# Autodesk Inventor assembly: Assembly
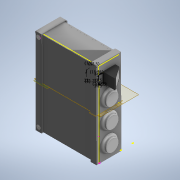
[picture p0: Inventor's stored thumbnail of the model, 180x180]
Saved by Autodesk Inventor 2020.1 (Build 241239000, 239)
## iProperties
Created: 2019-06-27
Part Number: Assembly
Document SubType Name: Assembly
Designer: jjsch
Author: jjsch
## Documents named in this file (11)
- C:\Users\jjsch\Documents\IIT\Coffee Project\coffee-is-a-core-value\hardware\Assembly.iam
- C:\Users\jjsch\Documents\IIT\Coffee Project\coffee-is-a-core-value\hardware\cam bien van tay.ipt
- C:\Users\jjsch\Documents\IIT\Coffee Project\coffee-is-a-core-value\hardware\lower casing.ipt
- C:\Users\jjsch\Documents\IIT\Coffee Project\coffee-is-a-core-value\hardware\upper casing.ipt
- C:\Users\jjsch\Documents\IIT\Coffee Project\coffee-is-a-core-value\hardware\Arcade Button_30mm.ipt
- C:\Users\jjsch\Documents\IIT\Coffee Project\coffee-is-a-core-value\hardware\top_casing.ipt
- C:\Users\jjsch\Documents\IIT\Coffee Project\coffee-is-a-core-value\hardware\rfid_top.ipt
- C:\Users\jjsch\Documents\IIT\Coffee Project\coffee-is-a-core-value\hardware\top_latch.ipt
- C:\Users\jjsch\Documents\Inventor\Content Center Files\R2020\en-US\GB_T 6561\Screw GB_T 6561 M4 x 10.ipt
- C:\Users\jjsch\Documents\IIT\Coffee Project\coffee-is-a-core-value\hardware\backplate.ipt
- C:\Users\jjsch\Documents\IIT\Coffee Project\coffee-is-a-core-value\hardware\front ring part.ipt
## Components (19 placed, 10 different names)
1. cam bien van tay:1 — Mate:22, Mate:24, Mate:25
2. lower casing:1 — Mate:10, Flush:1, Flush:2, Mate:27, Rotational:5, Rotational:6, Rotational:7, Rotational:8
3. upper casing:1 — Mate:1, Mate:2, Mate:3, Mate:4, Mate:5, Mate:6, Mate:10, Flush:1, Flush:2, Mate:11, Flush:3, Flush:4, Mate:22, Mate:24, Mate:25, Mate:26, Mate:28, Mate:31
4. Arcade Button_30mm:1 — Mate:3, Mate:4
5. Arcade Button_30mm:2 — Mate:2, Mate:5
6. Arcade Button_30mm:3 — Mate:1, Mate:6
7. top_casing:1 — Mate:11, Flush:3, Flush:4, Mate:12, Flush:5, Flush:6, Mate:19, Rigid:1, Mate:29, Flush:13, Mate:30, Rotational:9, Rotational:10
8. rfid_top:1 — Mate:12, Flush:5, Flush:6
9. top_latch:1 — Mate:19, Mate:29, Flush:13
10. Tapping screw GB/T 6561 M4x10:1 — Rotational:4
11. Tapping screw GB/T 6561 M4x10:2 — Rotational:9
12. Tapping screw GB/T 6561 M4x10:3 — Rigid:1
13. Tapping screw GB/T 6561 M4x10:4 — Rotational:10
14. backplate:1 — Mate:26, Mate:27, Mate:28, Rotational:4
15. Tapping screw GB/T 6561 M4x10:5 — Rotational:5
16. Tapping screw GB/T 6561 M4x10:6 — Rotational:6
17. Tapping screw GB/T 6561 M4x10:7 — Rotational:8
18. Tapping screw GB/T 6561 M4x10:8 — Rotational:7
19. front ring part:1 — Mate:30, Mate:31
## Relationships (34: Mate 19, Flush 7, RevoluteJoint 7, WeldJoint 1)
- Mate:1: upper casing:1 ↔ Arcade Button_30mm:3
- Mate:2: upper casing:1 ↔ Arcade Button_30mm:2
- Mate:3: upper casing:1 ↔ Arcade Button_30mm:1
- Mate:4: upper casing:1 ↔ Arcade Button_30mm:1
- Mate:5: upper casing:1 ↔ Arcade Button_30mm:2
- Mate:6: upper casing:1 ↔ Arcade Button_30mm:3
- Mate:10: lower casing:1 ↔ upper casing:1
- Flush:1: lower casing:1 ↔ upper casing:1
- Flush:2: lower casing:1 ↔ upper casing:1
- Mate:11: upper casing:1 ↔ top_casing:1
- Flush:3: upper casing:1 ↔ top_casing:1
- Flush:4: upper casing:1 ↔ top_casing:1
- Mate:12: top_casing:1 ↔ rfid_top:1
- Flush:5: top_casing:1 ↔ rfid_top:1
- Flush:6: top_casing:1 ↔ rfid_top:1
- Mate:19: top_casing:1 ↔ top_latch:1
- Mate:22: cam bien van tay:1 ↔ upper casing:1
- Mate:24: cam bien van tay:1 ↔ upper casing:1
- Mate:25: cam bien van tay:1 ↔ upper casing:1
- Mate:26: upper casing:1 ↔ backplate:1
- Mate:27: lower casing:1 ↔ backplate:1
- Mate:28: upper casing:1 ↔ backplate:1
- Rotational:4 [RevoluteJoint] (-2.4 mm): Tapping screw GB/T 6561 M4x10:1 ↔ backplate:1
- Rigid:1 [WeldJoint] (-5 mm): top_casing:1 ↔ Tapping screw GB/T 6561 M4x10:3
- Rotational:5 [RevoluteJoint]: lower casing:1 ↔ Tapping screw GB/T 6561 M4x10:5
- Rotational:6 [RevoluteJoint] (1 mm): lower casing:1 ↔ Tapping screw GB/T 6561 M4x10:6
- Mate:29 (0.25 mm): top_casing:1 ↔ top_latch:1
- Flush:13: top_casing:1 ↔ top_latch:1
- Rotational:7 [RevoluteJoint]: lower casing:1 ↔ Tapping screw GB/T 6561 M4x10:8
- Rotational:8 [RevoluteJoint]: lower casing:1 ↔ Tapping screw GB/T 6561 M4x10:7
- Mate:30: top_casing:1 ↔ front ring part:1
- Mate:31: upper casing:1 ↔ front ring part:1
- Rotational:9 [RevoluteJoint]: top_casing:1 ↔ Tapping screw GB/T 6561 M4x10:2
- Rotational:10 [RevoluteJoint]: top_casing:1 ↔ Tapping screw GB/T 6561 M4x10:4
